# Autodesk Inventor assembly: GPS_IMUMount
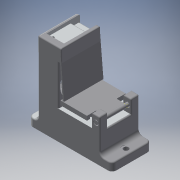
[picture p0: Inventor's stored thumbnail of the model, 180x180]
Saved by Autodesk Inventor 2016 (Build 200138000, 138)
## iProperties
Created: 2016-10-17
Part Number: GPS_IMUMount
Document SubType Name: Assembly
Designer: lachesis
Author: lachesis
## Documents named in this file (3)
- C:\Users\lachesis\git\Swarmathon-Robot\CAD-Files\PrintableSwarmie\GPS_IMUMount.iam
- C:\Users\lachesis\git\Swarmathon-Robot\CAD-Files\PrintableSwarmie\GPS_IMUMount.ipt
- C:\Users\lachesis\git\Swarmathon-Robot\CAD-Files\PrintableSwarmie\GPSDoor.ipt
## Components (2 placed, 2 different names)
1. GPS_IMUMount:1 — Rotational:1
2. GPSDoor:1 — Rotational:1
## Relationships (1: RevoluteJoint 1)
- Rotational:1 [RevoluteJoint]: GPS_IMUMount:1 ↔ GPSDoor:1
